# Autodesk Inventor assembly: FINAL
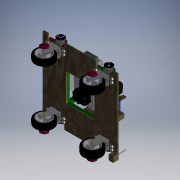
[picture p0: Inventor's stored thumbnail of the model, 180x180]
Saved by Autodesk Inventor 2016 (Build 200138000, 138)
## iProperties
Created: 2016-05-03
Part Number: FINAL
Document SubType Name: Assembly
Designer: Kenneth Daniel
Author: Kenneth Daniel
## Documents named in this file (81)
- E:\Dropbox\UMD\Spring 2016\ENES 100\CAD Drawings\Final assembly\FINAL.iam
- E:\Dropbox\UMD\Spring 2016\ENES 100\CAD Drawings\Final assembly\Milestone 8 & 9 Main Chasis.ipt
- E:\Dropbox\UMD\Spring 2016\ENES 100\CAD Drawings\Final assembly\Drive Motor.ipt
- E:\Dropbox\UMD\Spring 2016\ENES 100\CAD Drawings\Final assembly\Motor Mount.ipt
- E:\Dropbox\UMD\Spring 2016\ENES 100\CAD Drawings\Final assembly\EN ISO 7045 - M6 x 25 - 4.8 - H(3).ipt
- E:\Dropbox\UMD\Spring 2016\ENES 100\CAD Drawings\Final assembly\ISO 8673 - M8 x 1SFS-EN.ipt
- E:\Dropbox\UMD\Spring 2016\ENES 100\CAD Drawings\Final assembly\Main Motor to Sprocket Adapter.ipt
- E:\Dropbox\UMD\Spring 2016\ENES 100\CAD Drawings\Final assembly\Drive Motor_MIR.ipt
- E:\Dropbox\UMD\Spring 2016\ENES 100\CAD Drawings\Final assembly\Motor Mount_MIR.ipt
- E:\Dropbox\UMD\Spring 2016\ENES 100\CAD Drawings\Final assembly\Main Motor to Sprocket Adapter_MIR.ipt
- E:\Dropbox\UMD\Spring 2016\ENES 100\CAD Drawings\Final assembly\Drive Motor_MIR1.ipt
- E:\Dropbox\UMD\Spring 2016\ENES 100\CAD Drawings\Final assembly\Motor Mount_MIR1.ipt
- E:\Dropbox\UMD\Spring 2016\ENES 100\CAD Drawings\Final assembly\Main Motor to Sprocket Adapter_MIR1.ipt
- E:\Dropbox\UMD\Spring 2016\ENES 100\CAD Drawings\Final assembly\Drive Motor_MIR_MIR.ipt
- E:\Dropbox\UMD\Spring 2016\ENES 100\CAD Drawings\Final assembly\Motor Mount_MIR_MIR.ipt
- E:\Dropbox\UMD\Spring 2016\ENES 100\CAD Drawings\Final assembly\Main Motor to Sprocket Adapter_MIR_MIR.ipt
- E:\Dropbox\UMD\Spring 2016\ENES 100\CAD Drawings\Final assembly\Lifting Chasis.iam
- E:\Dropbox\UMD\Spring 2016\ENES 100\CAD Drawings\Final assembly\Axel Ending.ipt
- E:\Dropbox\UMD\Spring 2016\ENES 100\CAD Drawings\Final assembly\Axel Ending_MIR.ipt
- E:\Dropbox\UMD\Spring 2016\ENES 100\CAD Drawings\Final assembly\Axel Ending_MIR1.ipt
- E:\Dropbox\UMD\Spring 2016\ENES 100\CAD Drawings\Final assembly\Axel Ending_MIR_MIR.ipt
- E:\Dropbox\UMD\Spring 2016\ENES 100\CAD Drawings\Final assembly\Lifting Platform Assembly.iam
- E:\Dropbox\UMD\Spring 2016\ENES 100\CAD Drawings\Final assembly\Small Sprocket.ipt
- E:\Dropbox\UMD\Spring 2016\ENES 100\CAD Drawings\Final assembly\AS 1427 - M3.5 x 8(6) III.ipt
- E:\Dropbox\UMD\Spring 2016\ENES 100\CAD Drawings\Final assembly\Small Sprocket_MIR.ipt
- E:\Dropbox\UMD\Spring 2016\ENES 100\CAD Drawings\Final assembly\Small Sprocket_MIR1.ipt
- E:\Dropbox\UMD\Spring 2016\ENES 100\CAD Drawings\Final assembly\Small Sprocket_MIR_MIR.ipt
- E:\Dropbox\UMD\Spring 2016\ENES 100\CAD Drawings\Final assembly\arduino uno.iam
- E:\Dropbox\UMD\Spring 2016\ENES 100\CAD Drawings\Final assembly\Ponte H (PRONTO) (1).ipt
- E:\Dropbox\UMD\Spring 2016\ENES 100\CAD Drawings\Final assembly\Battery.ipt
- E:\Dropbox\UMD\Spring 2016\ENES 100\CAD Drawings\Final assembly\Circuit Board.ipt
- E:\Dropbox\UMD\Spring 2016\ENES 100\CAD Drawings\Final assembly\APC 220.ipt
- E:\Dropbox\UMD\Spring 2016\ENES 100\CAD Drawings\Final assembly\H Bridge #2.ipt
- E:\Dropbox\UMD\Spring 2016\ENES 100\CAD Drawings\Final assembly\Ultra Sonic Sensor.ipt
- E:\Dropbox\UMD\Spring 2016\ENES 100\CAD Drawings\Final assembly\Ultra Sonic Sensor Mounting.ipt
- E:\Dropbox\UMD\Spring 2016\ENES 100\CAD Drawings\Final assembly\Riser.ipt
- E:\Dropbox\UMD\Spring 2016\ENES 100\CAD Drawings\Final assembly\Riser_MIR.ipt
- E:\Dropbox\UMD\Spring 2016\ENES 100\CAD Drawings\Final assembly\Ultra Sonic Sensor Mounting_MIR.ipt
- E:\Dropbox\UMD\Spring 2016\ENES 100\CAD Drawings\Final assembly\Ultra Sonic Sensor_MIR.ipt
- E:\Dropbox\UMD\Spring 2016\ENES 100\CAD Drawings\Final assembly\Solenoid Interior.ipt
- E:\Dropbox\UMD\Spring 2016\ENES 100\CAD Drawings\Final assembly\Solonoid Outside.ipt
- E:\Dropbox\UMD\Spring 2016\ENES 100\CAD Drawings\Final assembly\Solenoid Mount.ipt
- E:\Dropbox\UMD\Spring 2016\ENES 100\CAD Drawings\Final assembly\Steel Rod.ipt
- E:\Dropbox\UMD\Spring 2016\ENES 100\CAD Drawings\Final assembly\Syring Mount.ipt
- E:\Dropbox\UMD\Spring 2016\ENES 100\CAD Drawings\Final assembly\Small Syringe.ipt
- E:\Dropbox\UMD\Spring 2016\ENES 100\CAD Drawings\Final assembly\Large Syring Mount.ipt
- E:\Dropbox\UMD\Spring 2016\ENES 100\CAD Drawings\Final assembly\Step Motor.iam
- E:\Dropbox\UMD\Spring 2016\ENES 100\CAD Drawings\Final assembly\Step Motor Rod.ipt
- E:\Dropbox\UMD\Spring 2016\ENES 100\CAD Drawings\Final assembly\Thin Wheel Mount.ipt
- E:\Dropbox\UMD\Spring 2016\ENES 100\CAD Drawings\Final assembly\Wheel Axel.ipt
- E:\Dropbox\UMD\Spring 2016\ENES 100\CAD Drawings\Final assembly\Metal  Sheet.ipt
- E:\Dropbox\UMD\Spring 2016\ENES 100\CAD Drawings\Final assembly\Modified Sprocketing.ipt
- E:\Dropbox\UMD\Spring 2016\ENES 100\CAD Drawings\Final assembly\Thin Wheel Mount_MIR.ipt
- E:\Dropbox\UMD\Spring 2016\ENES 100\CAD Drawings\Final assembly\Wheel Axel_MIR.ipt
- E:\Dropbox\UMD\Spring 2016\ENES 100\CAD Drawings\Final assembly\Axel Ending_MIR2.ipt
- E:\Dropbox\UMD\Spring 2016\ENES 100\CAD Drawings\Final assembly\Metal  Sheet_MIR.ipt
- E:\Dropbox\UMD\Spring 2016\ENES 100\CAD Drawings\Final assembly\Modified Sprocketing_MIR.ipt
- E:\Dropbox\UMD\Spring 2016\ENES 100\CAD Drawings\Final assembly\OSV Specific Wheel.ipt
- E:\Dropbox\UMD\Spring 2016\ENES 100\CAD Drawings\Final assembly\OSV Specific Wheel #2.ipt
- E:\Dropbox\UMD\Spring 2016\ENES 100\CAD Drawings\Final assembly\AS 1427 - M6 x 16(6) III.ipt
- E:\Dropbox\UMD\Spring 2016\ENES 100\CAD Drawings\Final assembly\OSV Specific Wheel #2_MIR.ipt
- E:\Dropbox\UMD\Spring 2016\ENES 100\CAD Drawings\Final assembly\Thin Wheel Mount_MIR1.ipt
- E:\Dropbox\UMD\Spring 2016\ENES 100\CAD Drawings\Final assembly\Wheel Axel_MIR1.ipt
- E:\Dropbox\UMD\Spring 2016\ENES 100\CAD Drawings\Final assembly\Axel Ending_MIR3.ipt
- E:\Dropbox\UMD\Spring 2016\ENES 100\CAD Drawings\Final assembly\Metal  Sheet_MIR1.ipt
- E:\Dropbox\UMD\Spring 2016\ENES 100\CAD Drawings\Final assembly\Modified Sprocketing_MIR1.ipt
- E:\Dropbox\UMD\Spring 2016\ENES 100\CAD Drawings\Final assembly\Thin Wheel Mount_MIR_MIR.ipt
- E:\Dropbox\UMD\Spring 2016\ENES 100\CAD Drawings\Final assembly\Wheel Axel_MIR_MIR.ipt
- E:\Dropbox\UMD\Spring 2016\ENES 100\CAD Drawings\Final assembly\Axel Ending_MIR2_MIR.ipt
- E:\Dropbox\UMD\Spring 2016\ENES 100\CAD Drawings\Final assembly\Metal  Sheet_MIR_MIR.ipt
- E:\Dropbox\UMD\Spring 2016\ENES 100\CAD Drawings\Final assembly\Modified Sprocketing_MIR_MIR.ipt
- E:\Dropbox\UMD\Spring 2016\ENES 100\CAD Drawings\Final assembly\OSV Specific Wheel_MIR.ipt
- E:\Dropbox\UMD\Spring 2016\ENES 100\CAD Drawings\Final assembly\Ph Reader.ipt
- E:\Dropbox\UMD\Spring 2016\ENES 100\CAD Drawings\Final assembly\Larger Syringe.ipt
- E:\Dropbox\UMD\Spring 2016\ENES 100\CAD Drawings\Final assembly\Lifting Motor.ipt
- E:\Dropbox\UMD\Spring 2016\ENES 100\CAD Drawings\Final assembly\Lifting Shaft.ipt
- E:\Dropbox\UMD\Spring 2016\ENES 100\CAD Drawings\Final assembly\REEL.ipt
- E:\Dropbox\UMD\Spring 2016\ENES 100\CAD Drawings\Final assembly\Thin Wheel Tire.ipt
- E:\Dropbox\UMD\Spring 2016\ENES 100\CAD Drawings\Final assembly\Thin Wheel Tire_MIR.ipt
- E:\Dropbox\UMD\Spring 2016\ENES 100\CAD Drawings\Final assembly\Larger Tire.ipt
- E:\Dropbox\UMD\Spring 2016\ENES 100\CAD Drawings\Final assembly\Larger Tire_MIR.ipt
## Components (133 placed, 80 different names)
1. Milestone 8 & 9 Main Chasis:1 — Mate:10, Mate:11, Mate:12, Mate:13, Tangent:1, Mate:14, Mate:15, Mate:55, Flush:9, Flush:10, Mate:56, Flush:12, Mate:61, Flush:13, Mate:63, Flush:14, Mate:65, Flush:15, Mate:72, Mate:77, Mate:84, Flush:20, Flush:21, Mate:85, Mate:86, Flush:23, Mate:93, Mate:95, Mate:101, Flush:25, Insert:6, Mate:134, Flush:36
2. SFS EN ISO 7045 H M6 x 25 - 4.8 - H:2 — Mate:4, Mate:8, Mate:10
3. SFS EN ISO 7045 H M6 x 25 - 4.8 - H:1 — Mate:3, Mate:7, Mate:12
4. SFS EN ISO 7045 H M6 x 25 - 4.8 - H:4 — Mate:2, Mate:6, Mate:11, Mate:16
5. SFS EN ISO 7045 H M6 x 25 - 4.8 - H:3 — Mate:1, Mate:5, Mate:13, Mate:17
6. Drive Motor:2 — Mate:9, Flush:1, Tangent:1, Mate:18, Flush:2, Mate:78
7. Motor Mount:1 — Mate:1, Mate:2, Mate:3, Mate:4, Mate:5, Mate:6, Mate:7, Mate:8, Mate:9, Flush:1
8. SFS-EN 28673 M8 x 1:1 — Mate:14, Mate:16
9. SFS-EN 28673 M8 x 1:2 — Mate:15, Mate:17
10. SFS-EN 28673 M8 x 1:3
11. SFS-EN 28673 M8 x 1:4
12. Main Motor to Sprocket Adapter:1 — Mate:18, Flush:2
13. SFS EN ISO 7045 H M6 x 25 - 4.8 - H:5 — Mate:20, Mate:24
14. SFS EN ISO 7045 H M6 x 25 - 4.8 - H:6 — Mate:21, Mate:25
15. SFS EN ISO 7045 H M6 x 25 - 4.8 - H:7 — Mate:22, Mate:26, Mate:28
16. SFS EN ISO 7045 H M6 x 25 - 4.8 - H:8 — Mate:23, Mate:27, Mate:29
17. Drive Motor_MIR:1 — Flush:3, Mate:19, Flush:4, Mate:30
18. Motor Mount_MIR:1 — Flush:3, Mate:19, Mate:20, Mate:21, Mate:22, Mate:23, Mate:24, Mate:25, Mate:26, Mate:27, Mate:64
19. SFS-EN 28673 M8 x 1:5 — Mate:28
20. SFS-EN 28673 M8 x 1:6 — Mate:29
21. SFS-EN 28673 M8 x 1:7
22. SFS-EN 28673 M8 x 1:8
23. Main Motor to Sprocket Adapter_MIR:1 — Flush:4, Mate:30
24. SFS EN ISO 7045 H M6 x 25 - 4.8 - H:9 — Mate:32, Mate:36
25. SFS EN ISO 7045 H M6 x 25 - 4.8 - H:10 — Mate:33, Mate:37
26. SFS EN ISO 7045 H M6 x 25 - 4.8 - H:11 — Mate:34, Mate:38, Mate:40
27. SFS EN ISO 7045 H M6 x 25 - 4.8 - H:12 — Mate:35, Mate:39, Mate:41
28. Drive Motor_MIR1:1 — Flush:5, Mate:31, Flush:6, Mate:42, Mate:60
29. Motor Mount_MIR1:1 — Flush:5, Mate:31, Mate:32, Mate:33, Mate:34, Mate:35, Mate:36, Mate:37, Mate:38, Mate:39, Flush:24
30. SFS-EN 28673 M8 x 1:9 — Mate:40
31. SFS-EN 28673 M8 x 1:10 — Mate:41
32. SFS-EN 28673 M8 x 1:11
33. SFS-EN 28673 M8 x 1:12
34. Main Motor to Sprocket Adapter_MIR1:1 — Flush:6, Mate:42, Mate:58, Mate:59
35. SFS EN ISO 7045 H M6 x 25 - 4.8 - H:13 — Mate:46, Mate:50
36. SFS EN ISO 7045 H M6 x 25 - 4.8 - H:14 — Mate:45, Mate:49
37. SFS EN ISO 7045 H M6 x 25 - 4.8 - H:15 — Mate:44, Mate:48, Mate:52
38. SFS EN ISO 7045 H M6 x 25 - 4.8 - H:16 — Mate:43, Mate:47, Mate:53
39. Drive Motor_MIR_MIR:1 — Mate:51, Flush:7, Mate:54, Flush:8, Flush:26, Flush:27
40. Motor Mount_MIR_MIR:1 — Mate:43, Mate:44, Mate:45, Mate:46, Mate:47, Mate:48, Mate:49, Mate:50, Mate:51, Flush:7, Mate:62, Mate:75, Mate:76, Angle:1, Flush:37
41. SFS-EN 28673 M8 x 1:13 — Mate:52
42. SFS-EN 28673 M8 x 1:14 — Mate:53
43. SFS-EN 28673 M8 x 1:15
44. SFS-EN 28673 M8 x 1:16
45. Main Motor to Sprocket Adapter_MIR_MIR:1 — Mate:54, Flush:8
46. Lifting Chasis:1 [sub-assembly] — Mate:55, Flush:9, Flush:10, Tangent:2, Tangent:3, Flush:11, Mate:57, Mate:66, Flush:16, Mate:67, Mate:79, Mate:87, Mate:94, Mate:136, Flush:39, Mate:137
47. Axel Ending:1 — Tangent:2, Tangent:3, Flush:11
48. Axel Ending_MIR:1 — Mate:141
49. Axel Ending_MIR1:1
50. Axel Ending_MIR_MIR:1 — Mate:139
51. Lifting Platform Assembly:1 [sub-assembly] — Mate:56, Mate:57, Flush:12
52. Small Sprocket:1 — Mate:58, Mate:59, Mate:60, Insert:1, Insert:2
53. AS 1427 Z Raised - Metric M3.5 x 8:1 — Insert:2
54. AS 1427 Z Raised - Metric M3.5 x 8:2 — Insert:1
55. AS 1427 Z Raised - Metric M3.5 x 8:3
56. AS 1427 Z Raised - Metric M3.5 x 8:4
57. Small Sprocket_MIR:1
58. Small Sprocket_MIR1:1 — Insert:3, Insert:4
59. AS 1427 Z Raised - Metric M3.5 x 8:5 — Insert:3
60. AS 1427 Z Raised - Metric M3.5 x 8:6 — Insert:4
61. AS 1427 Z Raised - Metric M3.5 x 8:7
62. AS 1427 Z Raised - Metric M3.5 x 8:8
63. Small Sprocket_MIR_MIR:1
64. arduino uno:1 [sub-assembly] — Mate:61, Flush:13, Mate:62
65. Ponte H (PRONTO) (1):1 — Mate:63, Flush:14, Mate:64
66. Battery:1 — Mate:65, Flush:15
67. Circuit Board:1 — Mate:66, Flush:16, Mate:67, Mate:68, Flush:17
68. APC 220:1 — Mate:68, Flush:17
69. H Bridge #2:1 — Mate:77, Mate:78, Mate:79
70. Ultra Sonic Sensor:1 — Mate:69, Mate:70, Mate:71
71. Ultra Sonic Sensor Mounting:1 — Mate:69, Mate:70, Mate:71, Mate:73, Flush:18, Mate:74
72. Riser:1 — Mate:72, Mate:73, Flush:18, Mate:74, Mate:75, Mate:76, Angle:1
73. Riser_MIR:1
74. Ultra Sonic Sensor Mounting_MIR:1
75. Ultra Sonic Sensor_MIR:1
76. Solenoid Interior:1 — Mate:80, Flush:19
77. Solonoid Outside:1 — Mate:80, Flush:19, Mate:89, Mate:90, Mate:91
78. Riser_MIR:2 — Mate:84, Flush:20, Flush:21, Flush:22
79. Steel Rod:1 — Mate:85, Flush:22
80. Syring Mount:1 — Mate:86, Flush:23, Flush:24, Mate:88, Tangent:4, Tangent:5, Tangent:6, Mate:92, Angle:2
81. Solenoid Mount:1 — Mate:87, Mate:88, Mate:89, Mate:90, Mate:91
82. Small Syringe:1 — Tangent:4, Tangent:5, Tangent:6, Mate:92, Angle:2
83. Large Syring Mount:1 — Mate:93, Mate:94, Mate:95, Mate:96, Mate:97, Mate:135, Flush:38, Tangent:7
84. Step Motor:1 [sub-assembly] — Mate:96, Mate:97, Mate:98, Mate:99, Mate:100, Insert:8, Insert:9
85. Step Motor Rod:1 — Mate:98, Mate:99, Mate:100
86. Thin Wheel Mount:1 — Mate:101, Flush:25, Flush:26, Mate:102, Mate:117, Insert:5
87. Wheel Axel:1 — Mate:102, Flush:27, Mate:103, Flush:28, Mate:104, Mate:105, Mate:106, Mate:108, Flush:29, Mate:116
88. Axel Ending:2 — Mate:103, Flush:28
89. Metal  Sheet:1 — Mate:104, Mate:105, Mate:106, Mate:107
90. Modified Sprocketing:1 — Mate:107, Mate:108, Flush:29
91. Thin Wheel Mount_MIR:1 — Mate:109
92. Wheel Axel_MIR:1 — Mate:109, Flush:30, Mate:110, Mate:111, Mate:112, Mate:113, Flush:31, Mate:114
93. Axel Ending_MIR2:1 — Flush:30, Mate:110
94. Metal  Sheet_MIR:1 — Mate:111, Mate:112, Mate:113, Mate:115
95. Modified Sprocketing_MIR:1 — Flush:31, Mate:114, Mate:115
96. OSV Specific Wheel:1 — Mate:132, Mate:133, Mate:143, Flush:41
97. OSV Specific Wheel #2:1 — Mate:116, Mate:117, Mate:142, Flush:40
98. AS 1427 Z Raised - Metric M6 x 16:1 — Insert:5
99. AS 1427 Z Raised - Metric M6 x 16:2 — Insert:6
100. AS 1427 Z Raised - Metric M6 x 16:3
101. AS 1427 Z Raised - Metric M6 x 16:4
102. AS 1427 Z Raised - Metric M6 x 16:5
103. AS 1427 Z Raised - Metric M6 x 16:6
104. AS 1427 Z Raised - Metric M6 x 16:7
105. AS 1427 Z Raised - Metric M6 x 16:8
106. OSV Specific Wheel #2_MIR:1
107. Thin Wheel Mount_MIR1:1 — Mate:118, Insert:7
108. Wheel Axel_MIR1:1 — Mate:118, Flush:32, Mate:119, Mate:120, Mate:121, Mate:122, Flush:33, Mate:123
109. Axel Ending_MIR3:1 — Flush:32, Mate:119
110. Metal  Sheet_MIR1:1 — Mate:120, Mate:121, Mate:122, Mate:124
111. Modified Sprocketing_MIR1:1 — Flush:33, Mate:123, Mate:124
112. Thin Wheel Mount_MIR_MIR:1 — Mate:125, Mate:133
113. Wheel Axel_MIR_MIR:1 — Mate:125, Mate:126, Flush:34, Mate:127, Mate:128, Mate:129, Mate:131, Flush:35, Mate:132
114. Axel Ending_MIR2_MIR:1 — Mate:126, Flush:34
115. Metal  Sheet_MIR_MIR:1 — Mate:127, Mate:128, Mate:129, Mate:130
116. Modified Sprocketing_MIR_MIR:1 — Mate:130, Mate:131, Flush:35
117. AS 1427 Z Raised - Metric M6 x 16:9 — Insert:7
118. AS 1427 Z Raised - Metric M6 x 16:10
119. AS 1427 Z Raised - Metric M6 x 16:11
120. AS 1427 Z Raised - Metric M6 x 16:12
121. OSV Specific Wheel_MIR:1
122. Ph Reader:1 — Mate:134, Flush:36, Flush:37
123. Larger Syringe:1 — Mate:135, Flush:38, Tangent:7
124. AS 1427 Z Raised - Metric M3.5 x 8:9 — Insert:8
125. AS 1427 Z Raised - Metric M3.5 x 8:10 — Insert:9
126. Lifting Motor:1 — Mate:136, Flush:39, Mate:137, Insert:10
127. Lifting Shaft:1 — Insert:10, Mate:138, Mate:140
128. REEL:1 — Mate:140, Mate:141
129. REEL:2 — Mate:138, Mate:139
130. Thin Wheel Tire:1 — Mate:142, Flush:40
131. Thin Wheel Tire_MIR:1
132. Larger Tire:1 — Mate:143, Flush:41
133. Larger Tire_MIR:1
## Relationships (200: Mate 140, Flush 41, Insert 10, Tangent 7, Angle 2)
- Mate:1: SFS EN ISO 7045 H M6 x 25 - 4.8 - H:3 ↔ Motor Mount:1
- Mate:2: SFS EN ISO 7045 H M6 x 25 - 4.8 - H:4 ↔ Motor Mount:1
- Mate:3: SFS EN ISO 7045 H M6 x 25 - 4.8 - H:1 ↔ Motor Mount:1
- Mate:4: SFS EN ISO 7045 H M6 x 25 - 4.8 - H:2 ↔ Motor Mount:1
- Mate:5: SFS EN ISO 7045 H M6 x 25 - 4.8 - H:3 ↔ Motor Mount:1
- Mate:6: SFS EN ISO 7045 H M6 x 25 - 4.8 - H:4 ↔ Motor Mount:1
- Mate:7: SFS EN ISO 7045 H M6 x 25 - 4.8 - H:1 ↔ Motor Mount:1
- Mate:8: SFS EN ISO 7045 H M6 x 25 - 4.8 - H:2 ↔ Motor Mount:1
- Mate:9: Drive Motor:2 ↔ Motor Mount:1
- Mate:10: Milestone 8 & 9 Main Chasis:1 ↔ SFS EN ISO 7045 H M6 x 25 - 4.8 - H:2
- Mate:11: Milestone 8 & 9 Main Chasis:1 ↔ SFS EN ISO 7045 H M6 x 25 - 4.8 - H:4
- Mate:12: Milestone 8 & 9 Main Chasis:1 ↔ SFS EN ISO 7045 H M6 x 25 - 4.8 - H:1
- Mate:13: Milestone 8 & 9 Main Chasis:1 ↔ SFS EN ISO 7045 H M6 x 25 - 4.8 - H:3
- Flush:1 (0.5 mm): Drive Motor:2 ↔ Motor Mount:1
- Tangent:1: Milestone 8 & 9 Main Chasis:1 ↔ Drive Motor:2
- Mate:14: Milestone 8 & 9 Main Chasis:1 ↔ SFS-EN 28673 M8 x 1:1
- Mate:15: Milestone 8 & 9 Main Chasis:1 ↔ SFS-EN 28673 M8 x 1:2
- Mate:16: SFS EN ISO 7045 H M6 x 25 - 4.8 - H:4 ↔ SFS-EN 28673 M8 x 1:1
- Mate:17: SFS EN ISO 7045 H M6 x 25 - 4.8 - H:3 ↔ SFS-EN 28673 M8 x 1:2
- Mate:18: Drive Motor:2 ↔ Main Motor to Sprocket Adapter:1
- Flush:2 (3 mm): Drive Motor:2 ↔ Main Motor to Sprocket Adapter:1
- Flush:3 (0.5 mm): Drive Motor_MIR:1 ↔ Motor Mount_MIR:1
- Mate:19: Drive Motor_MIR:1 ↔ Motor Mount_MIR:1
- Mate:20: SFS EN ISO 7045 H M6 x 25 - 4.8 - H:5 ↔ Motor Mount_MIR:1
- Mate:21: SFS EN ISO 7045 H M6 x 25 - 4.8 - H:6 ↔ Motor Mount_MIR:1
- Mate:22: SFS EN ISO 7045 H M6 x 25 - 4.8 - H:7 ↔ Motor Mount_MIR:1
- Mate:23: SFS EN ISO 7045 H M6 x 25 - 4.8 - H:8 ↔ Motor Mount_MIR:1
- Mate:24: SFS EN ISO 7045 H M6 x 25 - 4.8 - H:5 ↔ Motor Mount_MIR:1
- Mate:25: SFS EN ISO 7045 H M6 x 25 - 4.8 - H:6 ↔ Motor Mount_MIR:1
- Mate:26: SFS EN ISO 7045 H M6 x 25 - 4.8 - H:7 ↔ Motor Mount_MIR:1
- Mate:27: SFS EN ISO 7045 H M6 x 25 - 4.8 - H:8 ↔ Motor Mount_MIR:1
- Mate:28: SFS EN ISO 7045 H M6 x 25 - 4.8 - H:7 ↔ SFS-EN 28673 M8 x 1:5
- Mate:29: SFS EN ISO 7045 H M6 x 25 - 4.8 - H:8 ↔ SFS-EN 28673 M8 x 1:6
- Flush:4 (3 mm): Drive Motor_MIR:1 ↔ Main Motor to Sprocket Adapter_MIR:1
- Mate:30: Drive Motor_MIR:1 ↔ Main Motor to Sprocket Adapter_MIR:1
- Flush:5 (0.5 mm): Drive Motor_MIR1:1 ↔ Motor Mount_MIR1:1
- Mate:31: Drive Motor_MIR1:1 ↔ Motor Mount_MIR1:1
- Mate:32: SFS EN ISO 7045 H M6 x 25 - 4.8 - H:9 ↔ Motor Mount_MIR1:1
- Mate:33: SFS EN ISO 7045 H M6 x 25 - 4.8 - H:10 ↔ Motor Mount_MIR1:1
- Mate:34: SFS EN ISO 7045 H M6 x 25 - 4.8 - H:11 ↔ Motor Mount_MIR1:1
- Mate:35: SFS EN ISO 7045 H M6 x 25 - 4.8 - H:12 ↔ Motor Mount_MIR1:1
- Mate:36: SFS EN ISO 7045 H M6 x 25 - 4.8 - H:9 ↔ Motor Mount_MIR1:1
- Mate:37: SFS EN ISO 7045 H M6 x 25 - 4.8 - H:10 ↔ Motor Mount_MIR1:1
- Mate:38: SFS EN ISO 7045 H M6 x 25 - 4.8 - H:11 ↔ Motor Mount_MIR1:1
- Mate:39: SFS EN ISO 7045 H M6 x 25 - 4.8 - H:12 ↔ Motor Mount_MIR1:1
- Mate:40: SFS EN ISO 7045 H M6 x 25 - 4.8 - H:11 ↔ SFS-EN 28673 M8 x 1:9
- Mate:41: SFS EN ISO 7045 H M6 x 25 - 4.8 - H:12 ↔ SFS-EN 28673 M8 x 1:10
- Flush:6 (3 mm): Drive Motor_MIR1:1 ↔ Main Motor to Sprocket Adapter_MIR1:1
- Mate:42: Drive Motor_MIR1:1 ↔ Main Motor to Sprocket Adapter_MIR1:1
- Mate:43: SFS EN ISO 7045 H M6 x 25 - 4.8 - H:16 ↔ Motor Mount_MIR_MIR:1
- Mate:44: SFS EN ISO 7045 H M6 x 25 - 4.8 - H:15 ↔ Motor Mount_MIR_MIR:1
- Mate:45: SFS EN ISO 7045 H M6 x 25 - 4.8 - H:14 ↔ Motor Mount_MIR_MIR:1
- Mate:46: SFS EN ISO 7045 H M6 x 25 - 4.8 - H:13 ↔ Motor Mount_MIR_MIR:1
- Mate:47: SFS EN ISO 7045 H M6 x 25 - 4.8 - H:16 ↔ Motor Mount_MIR_MIR:1
- Mate:48: SFS EN ISO 7045 H M6 x 25 - 4.8 - H:15 ↔ Motor Mount_MIR_MIR:1
- Mate:49: SFS EN ISO 7045 H M6 x 25 - 4.8 - H:14 ↔ Motor Mount_MIR_MIR:1
- Mate:50: SFS EN ISO 7045 H M6 x 25 - 4.8 - H:13 ↔ Motor Mount_MIR_MIR:1
- Mate:51: Drive Motor_MIR_MIR:1 ↔ Motor Mount_MIR_MIR:1
- Flush:7 (0.5 mm): Drive Motor_MIR_MIR:1 ↔ Motor Mount_MIR_MIR:1
- Mate:52: SFS EN ISO 7045 H M6 x 25 - 4.8 - H:15 ↔ SFS-EN 28673 M8 x 1:13
- Mate:53: SFS EN ISO 7045 H M6 x 25 - 4.8 - H:16 ↔ SFS-EN 28673 M8 x 1:14
- Mate:54: Drive Motor_MIR_MIR:1 ↔ Main Motor to Sprocket Adapter_MIR_MIR:1
- Flush:8 (3 mm): Drive Motor_MIR_MIR:1 ↔ Main Motor to Sprocket Adapter_MIR_MIR:1
- Mate:55: Milestone 8 & 9 Main Chasis:1 ↔ Lifting Chasis:1
- Flush:9: Milestone 8 & 9 Main Chasis:1 ↔ Lifting Chasis:1
- Flush:10: Milestone 8 & 9 Main Chasis:1 ↔ Lifting Chasis:1
- Tangent:2: Lifting Chasis:1 ↔ Axel Ending:1
- Tangent:3: Lifting Chasis:1 ↔ Axel Ending:1
- Flush:11: Lifting Chasis:1 ↔ Axel Ending:1
- Mate:56: Milestone 8 & 9 Main Chasis:1 ↔ Lifting Platform Assembly:1
- Mate:57: Lifting Chasis:1 ↔ Lifting Platform Assembly:1
- Flush:12: Milestone 8 & 9 Main Chasis:1 ↔ Lifting Platform Assembly:1
- Mate:58: Main Motor to Sprocket Adapter_MIR1:1 ↔ Small Sprocket:1
- Mate:59: Main Motor to Sprocket Adapter_MIR1:1 ↔ Small Sprocket:1
- Mate:60: Drive Motor_MIR1:1 ↔ Small Sprocket:1
- Insert:1: Small Sprocket:1 ↔ AS 1427 Z Raised - Metric M3.5 x 8:2
- Insert:2: Small Sprocket:1 ↔ AS 1427 Z Raised - Metric M3.5 x 8:1
- Insert:3: Small Sprocket_MIR1:1 ↔ AS 1427 Z Raised - Metric M3.5 x 8:5
- Insert:4: Small Sprocket_MIR1:1 ↔ AS 1427 Z Raised - Metric M3.5 x 8:6
- Mate:61: Milestone 8 & 9 Main Chasis:1 ↔ arduino uno:1
- Flush:13: Milestone 8 & 9 Main Chasis:1 ↔ arduino uno:1
- Mate:62 (90 mm): Motor Mount_MIR_MIR:1 ↔ arduino uno:1
- Mate:63: Milestone 8 & 9 Main Chasis:1 ↔ Ponte H (PRONTO) (1):1
- Flush:14 (20 mm): Milestone 8 & 9 Main Chasis:1 ↔ Ponte H (PRONTO) (1):1
- Mate:64 (5 mm): Motor Mount_MIR:1 ↔ Ponte H (PRONTO) (1):1
- Mate:65: Milestone 8 & 9 Main Chasis:1 ↔ Battery:1
- Flush:15: Milestone 8 & 9 Main Chasis:1 ↔ Battery:1
- Mate:66: Lifting Chasis:1 ↔ Circuit Board:1
- Flush:16: Lifting Chasis:1 ↔ Circuit Board:1
- Mate:67: Lifting Chasis:1 ↔ Circuit Board:1
- Mate:68: Circuit Board:1 ↔ APC 220:1
- Flush:17: Circuit Board:1 ↔ APC 220:1
- Mate:69: Ultra Sonic Sensor:1 ↔ Ultra Sonic Sensor Mounting:1
- Mate:70: Ultra Sonic Sensor:1 ↔ Ultra Sonic Sensor Mounting:1
- Mate:71: Ultra Sonic Sensor:1 ↔ Ultra Sonic Sensor Mounting:1
- Mate:72: Milestone 8 & 9 Main Chasis:1 ↔ Riser:1
- Mate:73: Ultra Sonic Sensor Mounting:1 ↔ Riser:1
- Flush:18: Ultra Sonic Sensor Mounting:1 ↔ Riser:1
- Mate:74: Ultra Sonic Sensor Mounting:1 ↔ Riser:1
- Mate:75 (-10 mm): Motor Mount_MIR_MIR:1 ↔ Riser:1
- Mate:76 (15 mm): Motor Mount_MIR_MIR:1 ↔ Riser:1
- Angle:1 (-45 deg): Motor Mount_MIR_MIR:1 ↔ Riser:1
- Mate:77: Milestone 8 & 9 Main Chasis:1 ↔ H Bridge #2:1
- Mate:78 (10 mm): Drive Motor:2 ↔ H Bridge #2:1
- Mate:79 (-65 mm): Lifting Chasis:1 ↔ H Bridge #2:1
- Mate:80: Solenoid Interior:1 ↔ Solonoid Outside:1
- Flush:19 (-15 mm): Solenoid Interior:1 ↔ Solonoid Outside:1
- Mate:84: Milestone 8 & 9 Main Chasis:1 ↔ Riser_MIR:2
- Flush:20: Milestone 8 & 9 Main Chasis:1 ↔ Riser_MIR:2
- Flush:21: Milestone 8 & 9 Main Chasis:1 ↔ Riser_MIR:2
- Mate:85: Milestone 8 & 9 Main Chasis:1 ↔ Steel Rod:1
- Flush:22: Riser_MIR:2 ↔ Steel Rod:1
- Mate:86: Milestone 8 & 9 Main Chasis:1 ↔ Syring Mount:1
- Flush:23: Milestone 8 & 9 Main Chasis:1 ↔ Syring Mount:1
- Flush:24 (103 mm): Motor Mount_MIR1:1 ↔ Syring Mount:1
- Mate:87 (5 mm): Lifting Chasis:1 ↔ Solenoid Mount:1
- Mate:88 (5 mm): Syring Mount:1 ↔ Solenoid Mount:1
- Mate:89: Solonoid Outside:1 ↔ Solenoid Mount:1
- Mate:90: Solonoid Outside:1 ↔ Solenoid Mount:1
- Mate:91: Solonoid Outside:1 ↔ Solenoid Mount:1
- Tangent:4: Syring Mount:1 ↔ Small Syringe:1
- Tangent:5: Syring Mount:1 ↔ Small Syringe:1
- Tangent:6: Syring Mount:1 ↔ Small Syringe:1
- Mate:92: Syring Mount:1 ↔ Small Syringe:1
- Angle:2 (0 deg): Syring Mount:1 ↔ Small Syringe:1
- Mate:93: Milestone 8 & 9 Main Chasis:1 ↔ Large Syring Mount:1
- Mate:94: Lifting Chasis:1 ↔ Large Syring Mount:1
- Mate:95: Milestone 8 & 9 Main Chasis:1 ↔ Large Syring Mount:1
- Mate:96: Large Syring Mount:1 ↔ Step Motor:1
- Mate:97: Large Syring Mount:1 ↔ Step Motor:1
- Mate:98: Step Motor:1 ↔ Step Motor Rod:1
- Mate:99: Step Motor:1 ↔ Step Motor Rod:1
- Mate:100 (-15 mm): Step Motor:1 ↔ Step Motor Rod:1
- Mate:101: Milestone 8 & 9 Main Chasis:1 ↔ Thin Wheel Mount:1
- Flush:25: Milestone 8 & 9 Main Chasis:1 ↔ Thin Wheel Mount:1
- Flush:26: Drive Motor_MIR_MIR:1 ↔ Thin Wheel Mount:1
- Mate:102: Thin Wheel Mount:1 ↔ Wheel Axel:1
- Flush:27: Drive Motor_MIR_MIR:1 ↔ Wheel Axel:1
- Mate:103: Wheel Axel:1 ↔ Axel Ending:2
- Flush:28: Wheel Axel:1 ↔ Axel Ending:2
- Mate:104: Wheel Axel:1 ↔ Metal  Sheet:1
- Mate:105: Wheel Axel:1 ↔ Metal  Sheet:1
- Mate:106: Wheel Axel:1 ↔ Metal  Sheet:1
- Mate:107: Metal  Sheet:1 ↔ Modified Sprocketing:1
- Mate:108: Wheel Axel:1 ↔ Modified Sprocketing:1
- Flush:29 (-5 mm): Wheel Axel:1 ↔ Modified Sprocketing:1
- Mate:109: Thin Wheel Mount_MIR:1 ↔ Wheel Axel_MIR:1
- Flush:30: Wheel Axel_MIR:1 ↔ Axel Ending_MIR2:1
- Mate:110: Wheel Axel_MIR:1 ↔ Axel Ending_MIR2:1
- Mate:111: Wheel Axel_MIR:1 ↔ Metal  Sheet_MIR:1
- Mate:112: Wheel Axel_MIR:1 ↔ Metal  Sheet_MIR:1
- Mate:113: Wheel Axel_MIR:1 ↔ Metal  Sheet_MIR:1
- Flush:31 (-5 mm): Wheel Axel_MIR:1 ↔ Modified Sprocketing_MIR:1
- Mate:114: Wheel Axel_MIR:1 ↔ Modified Sprocketing_MIR:1
- Mate:115: Metal  Sheet_MIR:1 ↔ Modified Sprocketing_MIR:1
- Mate:116: Wheel Axel:1 ↔ OSV Specific Wheel #2:1
- Mate:117 (5 mm): Thin Wheel Mount:1 ↔ OSV Specific Wheel #2:1
- Insert:5: Thin Wheel Mount:1 ↔ AS 1427 Z Raised - Metric M6 x 16:1
- Insert:6: Milestone 8 & 9 Main Chasis:1 ↔ AS 1427 Z Raised - Metric M6 x 16:2
- Mate:118: Thin Wheel Mount_MIR1:1 ↔ Wheel Axel_MIR1:1
- Flush:32: Wheel Axel_MIR1:1 ↔ Axel Ending_MIR3:1
- Mate:119: Wheel Axel_MIR1:1 ↔ Axel Ending_MIR3:1
- Mate:120: Wheel Axel_MIR1:1 ↔ Metal  Sheet_MIR1:1
- Mate:121: Wheel Axel_MIR1:1 ↔ Metal  Sheet_MIR1:1
- Mate:122: Wheel Axel_MIR1:1 ↔ Metal  Sheet_MIR1:1
- Flush:33 (-5 mm): Wheel Axel_MIR1:1 ↔ Modified Sprocketing_MIR1:1
- Mate:123: Wheel Axel_MIR1:1 ↔ Modified Sprocketing_MIR1:1
- Mate:124: Metal  Sheet_MIR1:1 ↔ Modified Sprocketing_MIR1:1
- Mate:125: Thin Wheel Mount_MIR_MIR:1 ↔ Wheel Axel_MIR_MIR:1
- Mate:126: Wheel Axel_MIR_MIR:1 ↔ Axel Ending_MIR2_MIR:1
- Flush:34: Wheel Axel_MIR_MIR:1 ↔ Axel Ending_MIR2_MIR:1
- Mate:127: Wheel Axel_MIR_MIR:1 ↔ Metal  Sheet_MIR_MIR:1
- Mate:128: Wheel Axel_MIR_MIR:1 ↔ Metal  Sheet_MIR_MIR:1
- Mate:129: Wheel Axel_MIR_MIR:1 ↔ Metal  Sheet_MIR_MIR:1
- Mate:130: Metal  Sheet_MIR_MIR:1 ↔ Modified Sprocketing_MIR_MIR:1
- Mate:131: Wheel Axel_MIR_MIR:1 ↔ Modified Sprocketing_MIR_MIR:1
- Flush:35 (-5 mm): Wheel Axel_MIR_MIR:1 ↔ Modified Sprocketing_MIR_MIR:1
- Insert:7: Thin Wheel Mount_MIR1:1 ↔ AS 1427 Z Raised - Metric M6 x 16:9
- Mate:132: OSV Specific Wheel:1 ↔ Wheel Axel_MIR_MIR:1
- Mate:133 (2 mm): OSV Specific Wheel:1 ↔ Thin Wheel Mount_MIR_MIR:1
- Mate:134: Milestone 8 & 9 Main Chasis:1 ↔ Ph Reader:1
- Flush:36 (15 mm): Milestone 8 & 9 Main Chasis:1 ↔ Ph Reader:1
- Flush:37 (10 mm): Motor Mount_MIR_MIR:1 ↔ Ph Reader:1
- Mate:135: Large Syring Mount:1 ↔ Larger Syringe:1
- Flush:38 (40 mm): Large Syring Mount:1 ↔ Larger Syringe:1
- Tangent:7 (1.75 mm): Large Syring Mount:1 ↔ Larger Syringe:1
- Insert:8 (-5 mm): Step Motor:1 ↔ AS 1427 Z Raised - Metric M3.5 x 8:9
- Insert:9 (-5 mm): Step Motor:1 ↔ AS 1427 Z Raised - Metric M3.5 x 8:10
- Mate:136: Lifting Chasis:1 ↔ Lifting Motor:1
- Flush:39 (-20 mm): Lifting Chasis:1 ↔ Lifting Motor:1
- Mate:137: Lifting Chasis:1 ↔ Lifting Motor:1
- Insert:10 (-5 mm): Lifting Motor:1 ↔ Lifting Shaft:1
- Mate:138: Lifting Shaft:1 ↔ REEL:2
- Mate:139: Axel Ending_MIR_MIR:1 ↔ REEL:2
- Mate:140: Lifting Shaft:1 ↔ REEL:1
- Mate:141: Axel Ending_MIR:1 ↔ REEL:1
- Mate:142: OSV Specific Wheel #2:1 ↔ Thin Wheel Tire:1
- Flush:40: OSV Specific Wheel #2:1 ↔ Thin Wheel Tire:1
- Mate:143: OSV Specific Wheel:1 ↔ Larger Tire:1
- Flush:41: OSV Specific Wheel:1 ↔ Larger Tire:1
